# Autodesk Inventor assembly: Motor Assembly
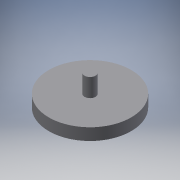
[picture p0: Inventor's stored thumbnail of the model, 180x180]
Saved by Autodesk Inventor 2016 (Build 200138000, 138)
## iProperties
Created: 2015-12-21
Part Number: Motor Assembly
Document SubType Name: Assembly
Designer: jonathan
Mass: 83.4941 g
Surface Area: 176.432 cm^2
Volume: 83.4941 cm^3
Density: 1 g/cm^3
Author: jonathan
## Documents named in this file (3)
- C:\Users\jonathan\Dropbox\Satellite\CAD\Motor Assembly.iam
- C:\Users\jonathan\Dropbox\Satellite\CAD\Brushless Motor.ipt
- C:\Users\jonathan\Dropbox\Satellite\CAD\Brushless Motor Shaft.ipt
## Components (2 placed, 2 different names)
1. Brushless Motor:1 — Insert:1
2. Brushless Motor Shaft:1 — Insert:1
## Relationships (1: Insert 1)
- Insert:1: Brushless Motor:1 ↔ Brushless Motor Shaft:1
